# Autodesk Inventor assembly: CustomRCAssembly
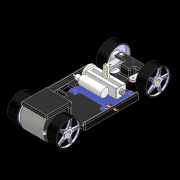
[picture p0: Inventor's stored thumbnail of the model, 180x180]
Saved by Autodesk Inventor 2022 (Build 260153000, 153)
## iProperties
Created: 2022-07-22
Part Number: CustomRCAssembly
Document SubType Name: Assembly
Designer: tandu
Author: tandu
## Documents named in this file (9)
- C:\Users\tandu\Documents\GrabCAD\Mini RCs\CustomRCAssembly.iam
- C:\Users\tandu\Documents\GrabCAD\Mini RCs\CustomChassis.ipt
- C:\Users\tandu\Documents\GrabCAD\Mini RCs\Linear Servo.ipt
- C:\Users\tandu\Documents\GrabCAD\Mini RCs\Ref STLs\Left_knuckle.ipt
- C:\Users\tandu\Documents\GrabCAD\Mini RCs\Custom_LeftKnuckle.ipt
- C:\Users\tandu\Documents\GrabCAD\Mini RCs\Custom_RightKnuckle.ipt
- C:\Users\tandu\Documents\GrabCAD\Mini RCs\Steering_BottomPlate.ipt
- C:\Users\tandu\Documents\GrabCAD\Mini RCs\N10 Motor DualShaftModded.ipt
- C:\Users\tandu\Documents\GrabCAD\Mini RCs\HW_back.ipt
## Components (11 placed, 8 different names)
1. CustomChassis:1 — Insert:1, Insert:2, Insert:3, Insert:4, Insert:5, Angle:1, Angle:2, Insert:6, Mate:1, Mate:2, Flush:1, Tangent:1
2. Linear Servo:1 — Insert:1, Insert:2
3. Left_knuckle:1 — Insert:3
4. Custom_LeftKnuckle:1 — Insert:4, Angle:2, Insert:10
5. Custom_RightKnuckle:1 — Insert:5, Angle:1, Insert:9
6. Steering_BottomPlate:1 — Insert:6, Mate:1
7. N10 Motor DualShaftModded:1 — Mate:2, Flush:1, Tangent:1, Insert:7, Insert:8
8. HW_back:1 — Insert:7
9. HW_back:2 — Insert:8
10. HW_back:3 — Insert:9
11. HW_back:4 — Insert:10
## Relationships (16: Insert 10, Angle 2, Mate 2, Flush 1, Tangent 1)
- Insert:1: CustomChassis:1 ↔ Linear Servo:1
- Insert:2: CustomChassis:1 ↔ Linear Servo:1
- Insert:3: CustomChassis:1 ↔ Left_knuckle:1
- Insert:4: CustomChassis:1 ↔ Custom_LeftKnuckle:1
- Insert:5: CustomChassis:1 ↔ Custom_RightKnuckle:1
- Angle:1 (0 deg): CustomChassis:1 ↔ Custom_RightKnuckle:1
- Angle:2 (0 deg): CustomChassis:1 ↔ Custom_LeftKnuckle:1
- Insert:6: CustomChassis:1 ↔ Steering_BottomPlate:1
- Mate:1: CustomChassis:1 ↔ Steering_BottomPlate:1
- Mate:2: CustomChassis:1 ↔ N10 Motor DualShaftModded:1
- Flush:1: CustomChassis:1 ↔ N10 Motor DualShaftModded:1
- Tangent:1: CustomChassis:1 ↔ N10 Motor DualShaftModded:1
- Insert:7: N10 Motor DualShaftModded:1 ↔ HW_back:1
- Insert:8: N10 Motor DualShaftModded:1 ↔ HW_back:2
- Insert:9: Custom_RightKnuckle:1 ↔ HW_back:3
- Insert:10: Custom_LeftKnuckle:1 ↔ HW_back:4
